# Autodesk Inventor assembly: leg1 _1_
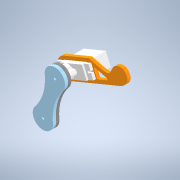
[picture p0: Inventor's stored thumbnail of the model, 180x180]
Saved by Autodesk Inventor 2020.3 (Build 243373000, 373)
## iProperties
Created: 2020-07-22
Part Number: leg1 _1_
Document SubType Name: Assembly
Designer: aditk
Author: aditk
## Documents named in this file (5)
- C:\Users\aditk\Desktop\PETcat\leg1 _1_.iam
- C:\Users\aditk\Desktop\PETcat\Part 6.ipt
- C:\Users\aditk\Desktop\PETcat\Part 7.ipt
- C:\Users\aditk\Desktop\PETcat\Part 18.ipt
- C:\Users\aditk\Desktop\PETcat\Part 1.ipt
## Components (4 placed, 4 different names)
1. Part 6:2 — Mate:1, Mate:2, Mate:3
2. Part 7:2 — Insert:1, Insert:2, Insert:3
3. Part 18:2 — Insert:1, Insert:2
4. Part 1:2 — Insert:3, Mate:1, Mate:2, Mate:3
## Relationships (6: Insert 3, Mate 3)
- Insert:1: Part 7:2 ↔ Part 18:2
- Insert:2: Part 7:2 ↔ Part 18:2
- Insert:3: Part 7:2 ↔ Part 1:2
- Mate:1: Part 6:2 ↔ Part 1:2
- Mate:2: Part 6:2 ↔ Part 1:2
- Mate:3: Part 6:2 ↔ Part 1:2
